# Autodesk Inventor assembly: fullbody
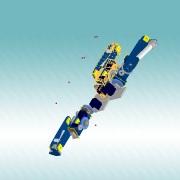
[picture p0: Inventor's stored thumbnail of the model, 180x180]
Saved by Autodesk Inventor 2020 (Build 240168000, 168)
## iProperties
Created: 2022-11-17
Part Number: fullbody
Document SubType Name: Assembly
Designer: kanazawakotaro
Author: kanazawakotaro
## Documents named in this file (3)
- C:\Users\金澤航太郎\Documents\Inventor\kamuy2\fullbody.iam
- C:\Users\金澤航太郎\Documents\Inventor\kamuy2\VER2.0.iam
- C:\Users\金澤航太郎\Documents\Inventor\kamuy2\VER2.0_MIR.iam
## Components (3 placed, 2 different names)
1. VER2.0:1 [sub-assembly] — メイト:1, フラッシュ:1
2. VER2.0:2 [sub-assembly] — メイト:1, フラッシュ:1
3. VER2.0_MIR:1 [sub-assembly]
## Relationships (2: Mate 1, Flush 1)
- メイト:1 [Mate]: VER2.0:1 ↔ VER2.0:2
- フラッシュ:1 [Flush]: VER2.0:1 ↔ VER2.0:2
